# Autodesk Inventor assembly: FRC Arena 2013 (TEST VERSION) - top rung - 26x28 arpan version
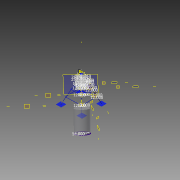
[picture p0: Inventor's stored thumbnail of the model, 180x180]
Saved by Autodesk Inventor 2013 (Build 170138000, 138)
## iProperties
Created: 2013-01-07
Part Number: FRC Arena 2013 (TEST VERSION) - top rung - 26x28 arpan version
Document SubType Name: Assembly
Designer: Phillip
Author: Phillip
## Documents named in this file (7)
- C:\Users\Arpan\Documents\GitHub\frc2013CAD\FIRST Arena 2013\FRC Arena 2013 (TEST VERSION) - top rung - 26x28 arpan version.iam
- C:\Users\Arpan\Documents\GitHub\frc2013CAD\FIRST Arena 2013\Arena\Arena Base.ipt
- C:\Users\Arpan\Documents\GitHub\frc2013CAD\FIRST Arena 2013\Pyramid\GE-13017.iam
- C:\Users\Arpan\Documents\GitHub\frc2013CAD\FIRST Arena 2013\Playing Configuration Constraint.ipt
- C:\Users\Arpan\Documents\GitHub\frc2013CAD\Robot Assembly - 6 wheel - toughbox mini - 26x28 official version.iam
- C:\Users\Arpan\Documents\GitHub\frc2013CAD\Cimber actual\Part4.ipt
- C:\Users\Arpan\Documents\GitHub\frc2013CAD\Cimber actual\Part5.ipt
## Components (7 placed, 6 different names)
1. Arena Base:1 — Mate:2, Angle:1, Mate:3, Angle:2, Flush:3
2. GE-13017:1 [sub-assembly] — Flush:5, Mate:5
3. Playing Configuration Constraint:1
4. Playing Configuration Constraint:2
5. Robot Assembly - 6 wheel - toughbox mini - 26x28 official version:1 [sub-assembly] — Flush:5, Mate:5, Mate:6, Angle:3, Flush:6, Flush:7, Flush:8, Flush:9
6. Part4:1 — Flush:6
7. Part5:1 — Flush:8, Flush:9
## Relationships (15: Flush 8, Mate 4, Angle 3)
- Mate:2: Arena Base:1
- Angle:1 (0 deg): Arena Base:1
- Flush:1 (2743.2 mm)
- Mate:3: Arena Base:1
- Angle:2 (0 deg): Arena Base:1
- Flush:2 (-2743.2 mm)
- Flush:3: Arena Base:1
- Flush:5: GE-13017:1 ↔ Robot Assembly - 6 wheel - toughbox mini - 26x28 official version:1
- Mate:5: GE-13017:1 ↔ Robot Assembly - 6 wheel - toughbox mini - 26x28 official version:1
- Mate:6: Robot Assembly - 6 wheel - toughbox mini - 26x28 official version:1
- Angle:3 (90 deg): Robot Assembly - 6 wheel - toughbox mini - 26x28 official version:1
- Flush:6: Robot Assembly - 6 wheel - toughbox mini - 26x28 official version:1 ↔ Part4:1
- Flush:7: Robot Assembly - 6 wheel - toughbox mini - 26x28 official version:1
- Flush:8: Robot Assembly - 6 wheel - toughbox mini - 26x28 official version:1 ↔ Part5:1
- Flush:9: Robot Assembly - 6 wheel - toughbox mini - 26x28 official version:1 ↔ Part5:1
